# Autodesk Inventor assembly: PRS- ASY Assembly1
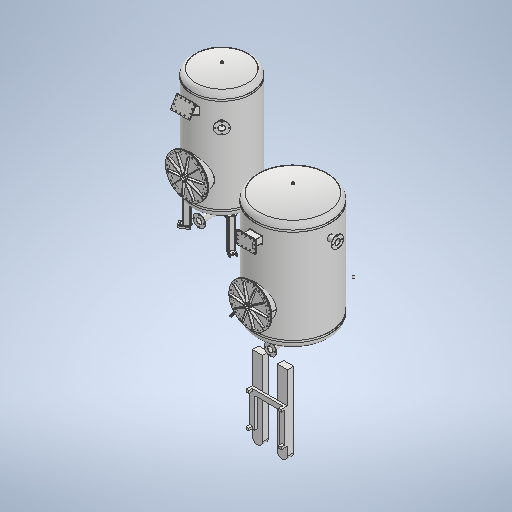
[picture p0: Inventor's stored thumbnail of the model, 512x512]
Saved by Autodesk Inventor 2026.2 (Build 302298000, 298)
## iProperties
Created: 2026-05-15
Part Number: PRS- ASY Assembly1
Document SubType Name: Assembly
Designer: admin
Author: admin
## Documents named in this file (3)
- C:\Users\admin\Documents\Inventor\PRS-Purovsk\0 ASY PRS MAIN.iam
- C:\Users\admin\Documents\Inventor\PRS-Purovsk\ASY PRS 1 Filter column D940.iam
- C:\Users\admin\Documents\Inventor\PRS-Purovsk\ASY PRS 1 Filter column D940_1200.iam
## Components (2 placed, 2 different names)
1. ASY PRS 1 Filter column D940:1 [sub-assembly] — Flush:1
2. ASY PRS 1 Filter column D940_1200:1 [sub-assembly] — Flush:2
## Relationships (2: Flush 2)
- Flush:1: ASY PRS 1 Filter column D940:1
- Flush:2: ASY PRS 1 Filter column D940_1200:1
